# Autodesk Inventor assembly: N_core
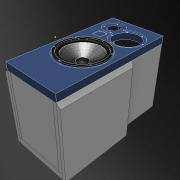
[picture p0: Inventor's stored thumbnail of the model, 180x180]
Saved by Autodesk Inventor 2022 (Build 260153070, 153G)
## iProperties
Created: 2021-11-16
Part Number: N_core
Document SubType Name: Assembly
Designer: kalugin_a
Mass: 16521.3 g
Surface Area: 21125.2 cm^2
Volume: 16521.3 cm^3
Density: 1 g/cm^3
Author: kalugin_a
## Documents named in this file (9)
- C:\Users\kalugin_a\Documents\Inventor\TUTO\MELAS\Workspace\N_core.iam
- C:\Users\kalugin_a\Documents\Inventor\TUTO\MELAS\Workspace\N_Front.ipt
- C:\Users\kalugin_a\Documents\Inventor\TUTO\MELAS\Workspace\N_into_side.ipt
- C:\Users\kalugin_a\Documents\Inventor\TUTO\MELAS\Workspace\N-Back_into.ipt
- C:\Users\kalugin_a\Documents\Inventor\TUTO\MELAS\Workspace\N_Bottom.ipt
- C:\Users\kalugin_a\Documents\Inventor\TUTO\MELAS\Workspace\MID.ipt
- C:\Users\kalugin_a\Documents\Inventor\TUTO\MELAS\Workspace\N__side_sticker.ipt
- C:\Users\kalugin_a\Documents\Inventor\TUTO\MELAS\Workspace\N__side_sticker_MIR.ipt
- C:\Users\kalugin_a\Documents\Inventor\TUTO\MELAS\Workspace\WOOFER.ipt
## Components (10 placed, 9 different names)
1. N_Front:1 — Жесткий:6
2. N_into_side:1 — Жесткий:2
3. N_into_side:2 — Жесткий:1
4. N-Back_into:1 — Жесткий:3, Жесткий:4, Жесткий:5
5. N_Flane_H — Жесткий:3
6. MID:1
7. N__side_sticker:1 — Жесткий:4
8. N__side_sticker_MIR:1 — Жесткий:5
9. N_Bottom:3 — Жесткий:1, Жесткий:2, Жесткий:6
10. WOOFER:2
## Relationships (6: WeldJoint 6)
- Жесткий:1 [WeldJoint]: N_into_side:2 ↔ N_Bottom:3
- Жесткий:2 [WeldJoint]: N_into_side:1 ↔ N_Bottom:3
- Жесткий:3 [WeldJoint]: N-Back_into:1 ↔ N_Flane_H
- Жесткий:4 [WeldJoint]: N-Back_into:1 ↔ N__side_sticker:1
- Жесткий:5 [WeldJoint]: N-Back_into:1 ↔ N__side_sticker_MIR:1
- Жесткий:6 [WeldJoint]: N_Front:1 ↔ N_Bottom:3
